# Autodesk Inventor assembly: Zespol1
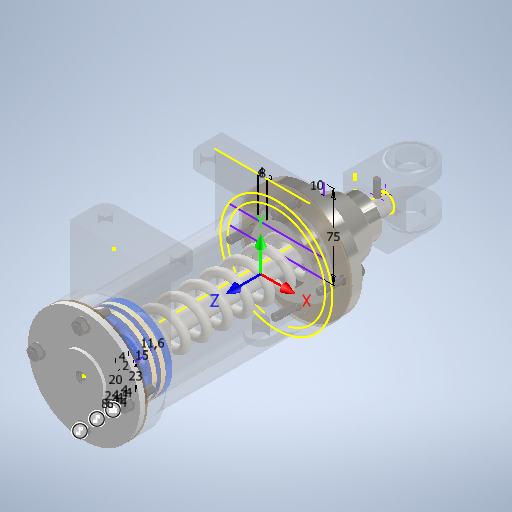
[picture p0: Inventor's stored thumbnail of the model, 512x512]
Saved by Autodesk Inventor 2025.2 (Build 292293000, 293)
## iProperties
Created: 2025-03-23
Part Number: Zespol1
Document SubType Name: Assembly
Designer: marci
Author: marci
## Documents named in this file (16)
- D:\Podstawy-Konstrukcji-Maszyn\Projekt1_temat21\nowe\Zespol1 (1).iam
- D:\Podstawy-Konstrukcji-Maszyn\Projekt1_temat21\nowe\01cylinder (2).ipt
- D:\Podstawy-Konstrukcji-Maszyn\Projekt1_temat21\nowe\02pokrywa.ipt
- D:\Podstawy-Konstrukcji-Maszyn\Projekt1_temat21\nowe\7Tłok.ipt
- D:\Podstawy-Konstrukcji-Maszyn\Projekt1_temat21\nowe\08pokrywa (2).ipt
- D:\Podstawy-Konstrukcji-Maszyn\Projekt1_temat21\nowe\06widelki.ipt
- D:\Podstawy-Konstrukcji-Maszyn\Projekt1_temat21\nowe\uszczelka.ipt
- D:\Podstawy-Konstrukcji-Maszyn\Projekt1_temat21\nowe\pierśnień.ipt
- D:\Podstawy-Konstrukcji-Maszyn\Projekt1_temat21\nowe\kołek.ipt
- D:\Podstawy-Konstrukcji-Maszyn\Projekt1_temat21\nowe\04tloczysko (3).ipt
- C:\Users\marci\Documents\repozytoria_git\Podstawy-Konstrukcji-Maszyn\Projekt1_temat21\content center\pl-PL\DIN 835\DIN 835 - M6 x 28 - 1.ipt
- C:\Users\marci\Documents\repozytoria_git\Podstawy-Konstrukcji-Maszyn\Projekt1_temat21\content center\pl-PL\DIN 988(1)\DIN 988 - S6 x 12.ipt
- C:\Users\marci\Documents\repozytoria_git\Podstawy-Konstrukcji-Maszyn\Projekt1_temat21\content center\pl-PL\DIN EN ISO 4032\DIN EN ISO 4032 - M6.ipt
- C:\Users\marci\Documents\repozytoria_git\Podstawy-Konstrukcji-Maszyn\Projekt1_temat21\content center\pl-PL\DIN EN ISO 4032\DIN EN ISO 4032 - M12.ipt
- D:\Podstawy-Konstrukcji-Maszyn\Projekt1_temat21\nowe\Sprężyna naciskowa12.ipt
- C:\Users\marci\Documents\repozytoria_git\Podstawy-Konstrukcji-Maszyn\Projekt1_temat21\content center\pl-PL\DIN 976-1 A\DIN 976-1 - M6 x 28 - A.ipt
## Components (38 placed, 15 different names)
1. 01cylinder (2):1 — Walcowe:3, Zestawiające:3, Walcowe:5, Zestawiające:7, Zestawiające:8, Obrotowe:14, Walcowe:8, Walcowe:9, Walcowe:10, Walcowe:11
2. 02pokrywa:1 — Obrotowe:27, Zestawiające:10, Obrotowe:28, Obrotowe:29, Obrotowe:30, Obrotowe:31
3. 7Tłok:1 — Obrotowe:15, Obrotowe:16, Obrotowe:17, Obrotowe:18, Równoległe:1
4. 08pokrywa (2):1 — Walcowe:4, Zestawiające:4, Walcowe:7, Obrotowe:1, Obrotowe:10, Obrotowe:11, Obrotowe:12, Obrotowe:13
5. 06widelki:1 — Walcowe:1, Zestawiające:1, Walcowe:2, Zestawiające:2, Obrotowe:13
6. uszczelka:1 — Obrotowe:14, Obrotowe:27
7. uszczelka:2 — Walcowe:3, Walcowe:4, Zestawiające:3, Zestawiające:4, Walcowe:6
8. pierśnień:1 — Obrotowe:15
9. pierśnień:2 — Obrotowe:16
10. kołek:1 — Walcowe:2, Zestawiające:2
11. 04tloczysko (3):2 — Walcowe:1, Zestawiające:1, Obrotowe:17, Zestawiające:9
12. DIN 835 M6 x 28:3 — Walcowe:5, Walcowe:6, Walcowe:7, Obrotowe:2
13. DIN 835 M6 x 28:4
14. DIN 988 S6 x 12:1 — Obrotowe:1, Obrotowe:3
15. DIN EN ISO 4032 M6:3 — Obrotowe:2, Obrotowe:3
16. DIN 835 M6 x 28:5
17. DIN 988 S6 x 12:2 — Obrotowe:10
18. DIN EN ISO 4032 M6:4
19. DIN 835 M6 x 28:6
20. DIN 988 S6 x 12:3 — Obrotowe:11
21. DIN EN ISO 4032 M6:5
22. DIN 835 M6 x 28:7
23. DIN 988 S6 x 12:4 — Obrotowe:12
24. DIN EN ISO 4032 M6:6
25. DIN EN ISO 4032 M12:1 — Obrotowe:18
26. Sprężyna naciskowa1:1 — Zestawiające:9, Równoległe:1
27. DIN 988 S6 x 12:5 — Obrotowe:29
28. DIN EN ISO 4032 M6:7
29. DIN 988 S6 x 12:6 — Obrotowe:28
30. DIN EN ISO 4032 M6:8
31. DIN 988 S6 x 12:7 — Obrotowe:30
32. DIN EN ISO 4032 M6:9
33. DIN 988 S6 x 12:8 — Obrotowe:31
34. DIN EN ISO 4032 M6:10
35. DIN 976-1 A M6 x 28:1 — Walcowe:8, Zestawiające:10
36. DIN 976-1 A M6 x 28:2 — Walcowe:9
37. DIN 976-1 A M6 x 28:3 — Walcowe:10
38. DIN 976-1 A M6 x 28:4 — Walcowe:11
## Relationships (47: RevoluteJoint 27, CylindricalJoint 11, Mate 8, Flush 1)
- Walcowe:1 [CylindricalJoint]: 06widelki:1 ↔ 04tloczysko (3):2
- Zestawiające:1 [Mate]: 06widelki:1 ↔ 04tloczysko (3):2
- Walcowe:2 [CylindricalJoint]: 06widelki:1 ↔ kołek:1
- Zestawiające:2 [Mate]: 06widelki:1 ↔ kołek:1
- Walcowe:3 [CylindricalJoint]: 01cylinder (2):1 ↔ uszczelka:2
- Walcowe:4 [CylindricalJoint]: 08pokrywa (2):1 ↔ uszczelka:2
- Zestawiające:3 [Mate]: 01cylinder (2):1 ↔ uszczelka:2
- Zestawiające:4 [Mate]: 08pokrywa (2):1 ↔ uszczelka:2
- Walcowe:5 [CylindricalJoint]: 01cylinder (2):1 ↔ DIN 835 M6 x 28:3
- Zestawiające:7 [Mate]: 01cylinder (2):1
- Zestawiające:8 [Mate]: 01cylinder (2):1
- Walcowe:6 [CylindricalJoint]: uszczelka:2 ↔ DIN 835 M6 x 28:3
- Walcowe:7 [CylindricalJoint]: 08pokrywa (2):1 ↔ DIN 835 M6 x 28:3
- Obrotowe:1 [RevoluteJoint]: 08pokrywa (2):1 ↔ DIN 988 S6 x 12:1
- Obrotowe:2 [RevoluteJoint]: DIN 835 M6 x 28:3 ↔ DIN EN ISO 4032 M6:3
- Obrotowe:3 [RevoluteJoint]: DIN 988 S6 x 12:1 ↔ DIN EN ISO 4032 M6:3
- [RevoluteJoint]: DIN 835 M6 x 28:5 ↔ DIN EN ISO 4032 M6:4
- [RevoluteJoint]: DIN 988 S6 x 12:2 ↔ DIN EN ISO 4032 M6:4
- [RevoluteJoint]: DIN 835 M6 x 28:6 ↔ DIN EN ISO 4032 M6:5
- [RevoluteJoint]: DIN 988 S6 x 12:3 ↔ DIN EN ISO 4032 M6:5
- [RevoluteJoint]: DIN 835 M6 x 28:7 ↔ DIN EN ISO 4032 M6:6
- [RevoluteJoint]: DIN 988 S6 x 12:4 ↔ DIN EN ISO 4032 M6:6
- Obrotowe:10 [RevoluteJoint]: 08pokrywa (2):1 ↔ DIN 988 S6 x 12:2
- Obrotowe:11 [RevoluteJoint]: 08pokrywa (2):1 ↔ DIN 988 S6 x 12:3
- Obrotowe:12 [RevoluteJoint]: 08pokrywa (2):1 ↔ DIN 988 S6 x 12:4
- Obrotowe:13 [RevoluteJoint]: 08pokrywa (2):1 ↔ 06widelki:1
- Obrotowe:14 [RevoluteJoint]: 01cylinder (2):1 ↔ uszczelka:1
- Obrotowe:15 [RevoluteJoint]: 7Tłok:1 ↔ pierśnień:1
- Obrotowe:16 [RevoluteJoint]: 7Tłok:1 ↔ pierśnień:2
- Obrotowe:17 [RevoluteJoint]: 7Tłok:1 ↔ 04tloczysko (3):2
- Obrotowe:18 [RevoluteJoint]: 7Tłok:1 ↔ DIN EN ISO 4032 M12:1
- Zestawiające:9 [Mate]: 04tloczysko (3):2 ↔ Sprężyna naciskowa1:1
- Równoległe:1 [Flush]: 7Tłok:1 ↔ Sprężyna naciskowa1:1
- [RevoluteJoint]: DIN 988 S6 x 12:5 ↔ DIN EN ISO 4032 M6:7
- [RevoluteJoint]: DIN 988 S6 x 12:6 ↔ DIN EN ISO 4032 M6:8
- [RevoluteJoint]: DIN 988 S6 x 12:7 ↔ DIN EN ISO 4032 M6:9
- [RevoluteJoint]: DIN 988 S6 x 12:8 ↔ DIN EN ISO 4032 M6:10
- Obrotowe:27 [RevoluteJoint]: 02pokrywa:1 ↔ uszczelka:1
- Walcowe:8 [CylindricalJoint]: 01cylinder (2):1 ↔ DIN 976-1 A M6 x 28:1
- Walcowe:9 [CylindricalJoint]: 01cylinder (2):1 ↔ DIN 976-1 A M6 x 28:2
- Walcowe:10 [CylindricalJoint]: 01cylinder (2):1 ↔ DIN 976-1 A M6 x 28:3
- Walcowe:11 [CylindricalJoint]: 01cylinder (2):1 ↔ DIN 976-1 A M6 x 28:4
- Zestawiające:10 [Mate]: 02pokrywa:1 ↔ DIN 976-1 A M6 x 28:1
- Obrotowe:28 [RevoluteJoint]: 02pokrywa:1 ↔ DIN 988 S6 x 12:6
- Obrotowe:29 [RevoluteJoint]: 02pokrywa:1 ↔ DIN 988 S6 x 12:5
- Obrotowe:30 [RevoluteJoint]: 02pokrywa:1 ↔ DIN 988 S6 x 12:7
- Obrotowe:31 [RevoluteJoint]: 02pokrywa:1 ↔ DIN 988 S6 x 12:8
## Named parameters: d119_d115 = 0 mm, d120_d116 = 161.782084 deg, d121_d117 = 0 mm, d122_d118 = 0 deg, d123_d115 = 0 mm, d124_d116 = 161.782084 deg, d125_d117 = 0 mm, d126_d118 = 0 deg, d127_d115 = 0 mm, d128_d116 = 161.782084 deg, d129_d117 = 0 mm, d130_d118 = 0 deg, d155_d117 = 0 mm, d156_d118 = 0 deg, d159_d117 = 0 mm, d160_d118 = 0 deg, d163_d117 = 0 mm, d164_d118 = 0 deg, d167_d117 = 0 mm, d168_d118 = 0 deg
